# Autodesk Inventor assembly: NASA-20-ARM
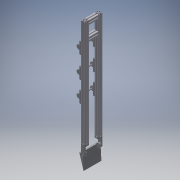
[picture p0: Inventor's stored thumbnail of the model, 180x180]
Saved by Autodesk Inventor 2019 (Build 230136000, 136)
## iProperties
Created: 2019-09-08
Part Number: NASA-20-ARM
Document SubType Name: Assembly
Designer: Rick Szalay
Author: Rick Szalay
## Documents named in this file (7)
- C:\Users\Rick Szalay\Documents\Inventor\NASA 20\NASA-20\ARM\NASA-20-ARM.iam
- C:\Users\Rick Szalay\Documents\Inventor\NASA 20\NASA-20\ARM\NASA-20-ARM-BA-01.ipt
- C:\Users\Rick Szalay\Documents\Inventor\NASA 20\NASA-20\ARM\NASA-20-ARM-BR-01.ipt
- C:\Users\Rick Szalay\Documents\Inventor\NASA 20\NASA-20\ARM\92981A230_ALLOY STEEL SHOULDER SCREW.ipt
- C:\Users\Rick Szalay\Documents\Inventor\NASA 20\NASA-20\ARM\NASA-20-ARM-CS-01.ipt
- C:\Users\Rick Szalay\Documents\Inventor\NASA 20\NASA-20\ARM\NASA-20-ARM-SH-01.ipt
- C:\Users\Rick Szalay\Documents\Inventor\NASA 20\NASA-20\ARM\NASA-20-ARM-HG-01.ipt
## Components (16 placed, 6 different names)
1. NASA-20-ARM-BA-01:1 — Flush:1, Flush:2, Mate:1, Mate:3, Flush:4, Mate:10, Flush:5, Mate:11, Flush:7, Flush:8, Mate:12, Flush:9, Mate:16, Flush:11, Mate:18, Flush:15, Flush:16
2. NASA-20-ARM-BA-01:2 — Flush:1, Flush:2, Mate:1, Flush:3, Mate:2, Flush:6, Flush:10, Flush:12, Mate:17, Flush:13, Flush:14
3. NASA-20-ARM-BR-01:1 — Flush:3, Mate:2, Mate:4, Mate:5, Mate:6
4. NASA-20-ARM-BR-01:2 — Mate:3, Flush:4, Mate:4
5. 92981A230_ALLOY STEEL SHOULDER SCREW:1 — Mate:5, Mate:6
6. NASA-20-ARM-BR-01:3 — Flush:6
7. NASA-20-ARM-BR-01:4 — Mate:10, Flush:5
8. 92981A230_ALLOY STEEL SHOULDER SCREW:2
9. NASA-20-ARM-CS-01:1 — Mate:11, Flush:7, Flush:8
10. NASA-20-ARM-CS-01:2 — Mate:12, Flush:9
11. NASA-20-ARM-BR-01:5 — Flush:10
12. NASA-20-ARM-BR-01:6 — Mate:16, Flush:11
13. 92981A230_ALLOY STEEL SHOULDER SCREW:3
14. NASA-20-ARM-SH-01:1 — Flush:12, Mate:19
15. NASA-20-ARM-HG-01:1 — Mate:17, Flush:13, Flush:14, Mate:19
16. NASA-20-ARM-HG-01:2 — Mate:18, Flush:15, Flush:16
## Relationships (35: Mate 19, Flush 16)
- Flush:1: NASA-20-ARM-BA-01:1 ↔ NASA-20-ARM-BA-01:2
- Flush:2: NASA-20-ARM-BA-01:1 ↔ NASA-20-ARM-BA-01:2
- Mate:1 (-127 mm): NASA-20-ARM-BA-01:1 ↔ NASA-20-ARM-BA-01:2
- Flush:3: NASA-20-ARM-BA-01:2 ↔ NASA-20-ARM-BR-01:1
- Mate:2: NASA-20-ARM-BA-01:2 ↔ NASA-20-ARM-BR-01:1
- Mate:3: NASA-20-ARM-BA-01:1 ↔ NASA-20-ARM-BR-01:2
- Flush:4: NASA-20-ARM-BA-01:1 ↔ NASA-20-ARM-BR-01:2
- Mate:4: NASA-20-ARM-BR-01:1 ↔ NASA-20-ARM-BR-01:2
- Mate:5: NASA-20-ARM-BR-01:1 ↔ 92981A230_ALLOY STEEL SHOULDER SCREW:1
- Mate:6: NASA-20-ARM-BR-01:1 ↔ 92981A230_ALLOY STEEL SHOULDER SCREW:1
- [Mate]: NASA-20-ARM-BR-01:3 ↔ NASA-20-ARM-BR-01:4
- [Mate]: NASA-20-ARM-BR-01:3 ↔ 92981A230_ALLOY STEEL SHOULDER SCREW:2
- [Mate]: NASA-20-ARM-BR-01:3 ↔ 92981A230_ALLOY STEEL SHOULDER SCREW:2
- Mate:10: NASA-20-ARM-BA-01:1 ↔ NASA-20-ARM-BR-01:4
- Flush:5: NASA-20-ARM-BA-01:1 ↔ NASA-20-ARM-BR-01:4
- Flush:6: NASA-20-ARM-BA-01:2 ↔ NASA-20-ARM-BR-01:3
- Mate:11: NASA-20-ARM-BA-01:1 ↔ NASA-20-ARM-CS-01:1
- Flush:7: NASA-20-ARM-BA-01:1 ↔ NASA-20-ARM-CS-01:1
- Flush:8: NASA-20-ARM-BA-01:1 ↔ NASA-20-ARM-CS-01:1
- Mate:12: NASA-20-ARM-BA-01:1 ↔ NASA-20-ARM-CS-01:2
- Flush:9: NASA-20-ARM-BA-01:1 ↔ NASA-20-ARM-CS-01:2
- [Mate]: NASA-20-ARM-BR-01:5 ↔ NASA-20-ARM-BR-01:6
- [Mate]: NASA-20-ARM-BR-01:5 ↔ 92981A230_ALLOY STEEL SHOULDER SCREW:3
- [Mate]: NASA-20-ARM-BR-01:5 ↔ 92981A230_ALLOY STEEL SHOULDER SCREW:3
- Mate:16: NASA-20-ARM-BA-01:1 ↔ NASA-20-ARM-BR-01:6
- Flush:10: NASA-20-ARM-BA-01:2 ↔ NASA-20-ARM-BR-01:5
- Flush:11: NASA-20-ARM-BA-01:1 ↔ NASA-20-ARM-BR-01:6
- Flush:12: NASA-20-ARM-BA-01:2 ↔ NASA-20-ARM-SH-01:1
- Mate:17: NASA-20-ARM-BA-01:2 ↔ NASA-20-ARM-HG-01:1
- Flush:13: NASA-20-ARM-BA-01:2 ↔ NASA-20-ARM-HG-01:1
- Flush:14: NASA-20-ARM-BA-01:2 ↔ NASA-20-ARM-HG-01:1
- Mate:18: NASA-20-ARM-BA-01:1 ↔ NASA-20-ARM-HG-01:2
- Flush:15: NASA-20-ARM-BA-01:1 ↔ NASA-20-ARM-HG-01:2
- Flush:16: NASA-20-ARM-BA-01:1 ↔ NASA-20-ARM-HG-01:2
- Mate:19: NASA-20-ARM-SH-01:1 ↔ NASA-20-ARM-HG-01:1
## Named parameters: d18_d16 = 0 mm, d19_d17 = 0 mm, d20_d13 = 0 mm, d29_d18_d16 = 0 mm, d30_d19_d17 = 0 mm, d31_d20_d13 = 0 mm
